# Autodesk Inventor assembly: Panel-Mprom
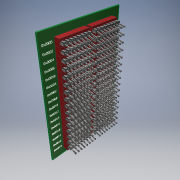
[picture p0: Inventor's stored thumbnail of the model, 180x180]
Saved by Autodesk Inventor 2018 (Build 220112000, 112)
## iProperties
Created: 2025-02-21
Part Number: Panel-Mprom
Material: Všeobecné
Document SubType Name: Assembly
Designer: Jozko Mrkvicka
Author: Jozko Mrkvicka
## Documents named in this file (4)
- D:\05_Projekty\Projects_Inventor\Haluska9000\Panel-Mprom.iam
- D:\05_Projekty\Projects_Inventor\Haluska9000\PCB\PCB#SwitchPanel.ipt
- D:\05_Projekty\Projects_Inventor\Haluska9000\PCB.ipt
- D:\05_Projekty\Projects_Inventor\Haluska9000\Switch.ipt
## Components (257 placed, 2 different names)
1. PCB#SwitchPanel:1 — Proti sobě:1, Stejný směr:1, Stejný směr:2, Proti sobě:2, Úhel:1, Proti sobě:3, Úhel:2, Proti sobě:4, Úhel:3, Proti sobě:5, Úhel:4, Souměrnost:2
2. Switch:1 — Proti sobě:1, Stejný směr:1, Stejný směr:2
3. Switch:2
4. Switch:3
5. Switch:4
6. Switch:5
7. Switch:6
8. Switch:7
9. Switch:8
10. Switch:9
11. Switch:10
12. Switch:11
13. Switch:12
14. Switch:13
15. Switch:14
16. Switch:15
17. Switch:16
18. Switch:17
19. Switch:18
20. Switch:19
21. Switch:20
22. Switch:21
23. Switch:22
24. Switch:23
25. Switch:24
26. Switch:25
27. Switch:26
28. Switch:27
29. Switch:28
30. Switch:29
31. Switch:30
32. Switch:31
33. Switch:32
34. Switch:33
35. Switch:34
36. Switch:35
37. Switch:36
38. Switch:37
39. Switch:38
40. Switch:39
41. Switch:40
42. Switch:41
43. Switch:42
44. Switch:43
45. Switch:44
46. Switch:45
47. Switch:46
48. Switch:47
49. Switch:48
50. Switch:49
51. Switch:50
52. Switch:51
53. Switch:52
54. Switch:53
55. Switch:54
56. Switch:55
57. Switch:56
58. Switch:57
59. Switch:58
60. Switch:59
61. Switch:60
62. Switch:61
63. Switch:62
64. Switch:63
65. Switch:64
66. Switch:65
67. Switch:66
68. Switch:67
69. Switch:68
70. Switch:69
71. Switch:70
72. Switch:71
73. Switch:72
74. Switch:73
75. Switch:74
76. Switch:75
77. Switch:76
78. Switch:77
79. Switch:78
80. Switch:79
81. Switch:80
82. Switch:81
83. Switch:82
84. Switch:83
85. Switch:84
86. Switch:85
87. Switch:86
88. Switch:87
89. Switch:88
90. Switch:89
91. Switch:90
92. Switch:91
93. Switch:92
94. Switch:93
95. Switch:94
96. Switch:95
97. Switch:96
98. Switch:97
99. Switch:98
100. Switch:99
101. Switch:100
102. Switch:101
103. Switch:102
104. Switch:103
105. Switch:104
106. Switch:105
107. Switch:106
108. Switch:107
109. Switch:108
110. Switch:109
111. Switch:110
112. Switch:111
113. Switch:112
114. Switch:113
115. Switch:114
116. Switch:115
117. Switch:116
118. Switch:117
119. Switch:118
120. Switch:119
121. Switch:120
122. Switch:121
123. Switch:122
124. Switch:123
125. Switch:124
126. Switch:125
127. Switch:126
128. Switch:127
129. Switch:128
130. Switch:129
131. Switch:130
132. Switch:131
133. Switch:132
134. Switch:133
135. Switch:134
136. Switch:135
137. Switch:136
138. Switch:137
139. Switch:138
140. Switch:139
141. Switch:140
142. Switch:141
143. Switch:142
144. Switch:143
145. Switch:144
146. Switch:145
147. Switch:146
148. Switch:147
149. Switch:148
150. Switch:149
151. Switch:150
152. Switch:151
153. Switch:152
154. Switch:153
155. Switch:154
156. Switch:155
157. Switch:156
158. Switch:157
159. Switch:158
160. Switch:159
161. Switch:160
162. Switch:161
163. Switch:162
164. Switch:163
165. Switch:164
166. Switch:165
167. Switch:166
168. Switch:167
169. Switch:168
170. Switch:169
171. Switch:170
172. Switch:171
173. Switch:172
174. Switch:173
175. Switch:174
176. Switch:175
177. Switch:176
178. Switch:177
179. Switch:178
180. Switch:179
181. Switch:180
182. Switch:181
183. Switch:182
184. Switch:183
185. Switch:184
186. Switch:185
187. Switch:186
188. Switch:187
189. Switch:188
190. Switch:189
191. Switch:190
192. Switch:191
193. Switch:192
194. Switch:193
195. Switch:194
196. Switch:195
197. Switch:196
198. Switch:197
199. Switch:198
200. Switch:199
201. Switch:200
202. Switch:201
203. Switch:202
204. Switch:203
205. Switch:204
206. Switch:205
207. Switch:206
208. Switch:207
209. Switch:208
210. Switch:209
211. Switch:210
212. Switch:211
213. Switch:212
214. Switch:213
215. Switch:214
216. Switch:215
217. Switch:216
218. Switch:217
219. Switch:218
220. Switch:219
221. Switch:220
222. Switch:221
223. Switch:222
224. Switch:223
225. Switch:224
226. Switch:225
227. Switch:226
228. Switch:227
229. Switch:228
230. Switch:229
231. Switch:230
232. Switch:231
233. Switch:232
234. Switch:233
235. Switch:234
236. Switch:235
237. Switch:236
238. Switch:237
239. Switch:238
240. Switch:239
241. Switch:240
242. Switch:241
243. Switch:242
244. Switch:243
245. Switch:244
246. Switch:245
247. Switch:246
248. Switch:247
249. Switch:248
250. Switch:249
251. Switch:250
252. Switch:251
253. Switch:252
254. Switch:253
255. Switch:254
256. Switch:255
257. Switch:256
## Component patterns: (2 elements), (128 elements, first: Switch:1), Pole komponent 1:2 (128 elements)
## Relationships (13: Mate 5, Angle 4, Flush 2, Symmetry 2)
- Proti sobě:1 [Mate]: PCB#SwitchPanel:1 ↔ Switch:1
- Stejný směr:1 [Flush] (12.7 mm): PCB#SwitchPanel:1 ↔ Switch:1
- Stejný směr:2 [Flush] (25.4 mm): PCB#SwitchPanel:1 ↔ Switch:1
- Proti sobě:2 [Mate]: PCB#SwitchPanel:1
- Úhel:1 [Angle] (0 deg): PCB#SwitchPanel:1
- Proti sobě:3 [Mate]: PCB#SwitchPanel:1
- Úhel:2 [Angle] (0 deg): PCB#SwitchPanel:1
- Souměrnost:1 [Symmetry]
- Proti sobě:4 [Mate]: PCB#SwitchPanel:1
- Úhel:3 [Angle] (0 deg): PCB#SwitchPanel:1
- Proti sobě:5 [Mate]: PCB#SwitchPanel:1
- Úhel:4 [Angle] (0 deg): PCB#SwitchPanel:1
- Souměrnost:2 [Symmetry]: PCB#SwitchPanel:1
## Named parameters: distanceVerticalBit = 12.7 mm, distanceHorizontalBit = 6.604 mm, countVertical = 16, countHorizontal = 8, pcbOffsetVertical = 12.7 mm, pcbOffsetHorizontal = 25.4 mm, distanceHorizontalBetweenBytes = 5.08 mm
